# Autodesk Inventor assembly: Ender-press
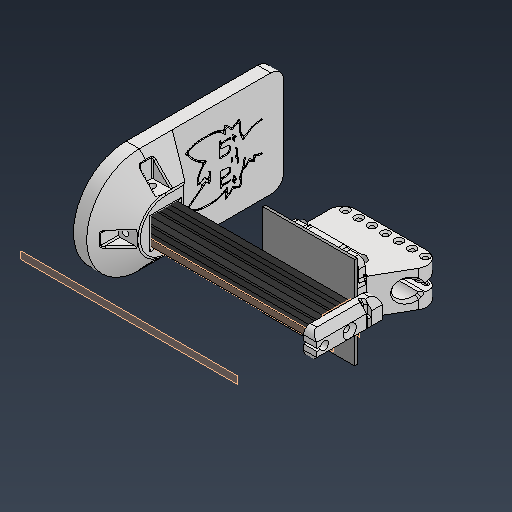
[picture p0: Inventor's stored thumbnail of the model, 512x512]
Saved by Autodesk Inventor 2026.2 (Build 302298010, 298A)
## iProperties
Created: 2026-06-05
Part Number: Ender-press
Document SubType Name: Assembly
Designer: szymo
Author: szymo
## Documents named in this file (6)
- D:\tech\github\Ender-press\3D\Ender-press.iam
- D:\tech\github\Ender-press\3D\2020.ipt
- D:\tech\github\Ender-press\3D\Base.ipt
- D:\tech\github\Ender-press\3D\Plateo.ipt
- D:\tech\github\Ender-press\3D\CAP.ipt
- D:\tech\github\Ender-press\3D\Soldering_iron_holder.ipt
## Components (5 placed, 5 different names)
1. 2020:1 — Flush:1, Flush:2, Flush:4, Flush:5, Flush:6, Flush:7, Flush:8, Flush:9, Flush:10
2. Base:1 — Flush:1, Flush:2, Flush:4, Flush:5, Flush:6
3. Plateo:1 — Flush:7, Flush:8, Flush:9, Flush:11, Flush:12
4. CAP:1 — Flush:10
5. Soldering_iron_holder:1 — Flush:11, Flush:12
## Relationships (11: Flush 11)
- Flush:1: 2020:1 ↔ Base:1
- Flush:2: 2020:1 ↔ Base:1
- Flush:4: 2020:1 ↔ Base:1
- Flush:5: 2020:1 ↔ Base:1
- Flush:6 (72.5 mm): 2020:1 ↔ Base:1
- Flush:7: 2020:1 ↔ Plateo:1
- Flush:8 (3.85 mm): 2020:1 ↔ Plateo:1
- Flush:9 (25 mm): 2020:1 ↔ Plateo:1
- Flush:10: 2020:1 ↔ CAP:1
- Flush:11: Plateo:1 ↔ Soldering_iron_holder:1
- Flush:12: Plateo:1 ↔ Soldering_iron_holder:1
